# Autodesk Inventor assembly: 2M2+wzmocnienie
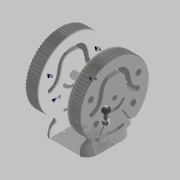
[picture p0: Inventor's stored thumbnail of the model, 180x180]
Saved by Autodesk Inventor 2021 (Build 250183000, 183)
## iProperties
Created: 2021-09-01
Part Number: 2M2+wzmocnienie
Document SubType Name: Assembly
Designer: marci
Author: marci
## Documents named in this file (7)
- C:\Users\marci\Desktop\Projekt ramienia\2M2\2M2+wzmocnienie.iam
- C:\Users\marci\Desktop\Projekt ramienia\2M2\Wzmocnienie 2M2.ipt
- C:\Users\marci\Desktop\Projekt ramienia\2M2\2M2MAedit.ipt
- C:\Users\marci\Desktop\Projekt ramienia\2M2\Tuleja środkowa.ipt
- C:\Users\marci\Desktop\Projekt ramienia\Nowy folder\pl-PL\ISO 4762(2)\ISO 4762 - M6 x 20ISO.ipt
- C:\Users\marci\Desktop\Projekt ramienia\Nowy folder\pl-PL\ISO 7091\ISO 7091 - ST 6 - 100 HV.ipt
- C:\Users\marci\Desktop\Projekt ramienia\Nowy folder\pl-PL\ISO 4036(2)\ISO 4036 - M6(2).ipt
## Components (7 placed, 6 different names)
1. Wzmocnienie 2M2:1 — Zestawiające:1, Zestawiające:2, Równoległe:1, Zestawiające:3, Zestawiające:4, Równoległe:2, Wstawiające:1
2. 2M2MAedit:1 — Zestawiające:3, Zestawiające:4, Równoległe:2
3. 2M2MAedit:2 — Zestawiające:1, Zestawiające:2, Równoległe:1
4. Tuleja środkowa:1 — Wstawiające:1
5. ISO 4762 M6 x 20:1
6. ISO 7091 ST 6 - 100 HV:1
7. ISO 4036 M6:1
## Relationships (7: Mate 4, Flush 2, Insert 1)
- Zestawiające:1 [Mate]: Wzmocnienie 2M2:1 ↔ 2M2MAedit:2
- Zestawiające:2 [Mate]: Wzmocnienie 2M2:1 ↔ 2M2MAedit:2
- Równoległe:1 [Flush]: Wzmocnienie 2M2:1 ↔ 2M2MAedit:2
- Zestawiające:3 [Mate]: Wzmocnienie 2M2:1 ↔ 2M2MAedit:1
- Zestawiające:4 [Mate]: Wzmocnienie 2M2:1 ↔ 2M2MAedit:1
- Równoległe:2 [Flush]: Wzmocnienie 2M2:1 ↔ 2M2MAedit:1
- Wstawiające:1 [Insert]: Wzmocnienie 2M2:1 ↔ Tuleja środkowa:1
